# Autodesk Inventor assembly: Montiert
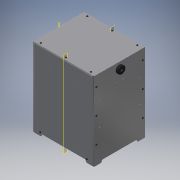
[picture p0: Inventor's stored thumbnail of the model, 180x180]
Saved by Autodesk Inventor 2018 (Build 220112000, 112)
## iProperties
Created: 2017-11-12
Part Number: Montiert
Material: Generisch
Document SubType Name: Assembly
## Documents named in this file (13)
- C:\git\RoKu-ProjectX01\Konstruktion\Montiert.iam
- C:\git\RoKu-ProjectX01\Konstruktion\Brenner.ipt
- C:\git\RoKu-ProjectX01\Konstruktion\Gegenhalter.ipt
- C:\git\RoKu-ProjectX01\Konstruktion\BrennerBrennTeil.ipt
- C:\git\RoKu-ProjectX01\Konstruktion\Back.ipt
- C:\git\RoKu-ProjectX01\Konstruktion\Seite.ipt
- C:\git\RoKu-ProjectX01\Konstruktion\Front.ipt
- C:\git\RoKu-ProjectX01\Konstruktion\Deckel.ipt
- C:\git\RoKu-ProjectX01\Konstruktion\MutterMitUScheibe.ipt
- C:\git\RoKu-ProjectX01\Konstruktion\BrennerHalter.ipt
- C:\Users\kuckal\Documents\Inventor\Content Center Files\R2018\de-DE\ISO 7380-1\ISO 7380-1 - M4 x 8.ipt
- C:\Users\kuckal\Documents\Inventor\Content Center Files\R2018\de-DE\ISO 7380-1\ISO 7380-1 - M4 x 6.ipt
- C:\Users\kuckal\Documents\Inventor\Content Center Files\R2018\de-DE\DIN EN 24 036(2)\DIN EN 24 036 - M4.ipt
## Components (65 placed, 12 different names)
1. Brenner:1 — Fluchtend:1, Fluchtend:2, Fluchtend:3, Passend:1, Passend:2, Fluchtend:4, Passend:3, Passend:4, Fluchtend:13, Fluchtend:14, Einfügen:37, Einfügen:38, Einfügen:39, Einfügen:40, Einfügen:41, Einfügen:42, Einfügen:43, Einfügen:44, Einfügen:45, Einfügen:46, Einfügen:47, Einfügen:48
2. Gegenhalter:1 — Passend:1, Passend:2, Einfügen:55, Einfügen:56, Einfügen:57, Einfügen:58, Einfügen:59, Einfügen:60, Einfügen:61, Einfügen:62, Einfügen:63, Einfügen:64, Einfügen:65, Einfügen:66
3. BrennerBrennTeil:1 — Fluchtend:4
4. Back:1 — Passend:3, Passend:4, Passend:5, Passend:6, Fluchtend:6, Fluchtend:7, Passend:7, Fluchtend:8, Fluchtend:9, Einfügen:25, Einfügen:26, Einfügen:27, Einfügen:28, Einfügen:29, Einfügen:30
5. Seite:1 — Passend:6, Fluchtend:6, Fluchtend:7, Passend:8, Fluchtend:11, Passend:9, Fluchtend:12, Passend:11, Passend:12, Passend:13, Passend:14, Einfügen:13, Einfügen:14, Einfügen:52, Einfügen:53, Einfügen:54
6. Seite:2 — Passend:7, Fluchtend:8, Fluchtend:9, Fluchtend:10, Passend:23, Passend:24, Passend:25, Passend:26, Einfügen:11, Einfügen:12, Einfügen:49, Einfügen:50, Einfügen:51
7. Front:1 — Passend:8, Fluchtend:10, Fluchtend:11, Passend:10, Einfügen:15, Einfügen:16, Einfügen:17, Einfügen:18, Einfügen:19, Einfügen:20
8. Deckel:1 — Passend:9, Fluchtend:12, Passend:10, Einfügen:31, Einfügen:32, Einfügen:33, Einfügen:34, Einfügen:35, Einfügen:36
9. MutterMitUScheibe:3 — Passend:23, Passend:24
10. MutterMitUScheibe:4 — Passend:25, Passend:26
11. MutterMitUScheibe:10 — Passend:11, Passend:12
12. MutterMitUScheibe:11 — Passend:13, Passend:14
13. BrennerHalter:1 — Fluchtend:13, Fluchtend:14
14. ISO 7380-1 M4 x 6:11 — Einfügen:11
15. ISO 7380-1 M4 x 6:12 — Einfügen:12
16. ISO 7380-1 M4 x 6:13 — Einfügen:13
17. ISO 7380-1 M4 x 6:14 — Einfügen:14
18. ISO 7380-1 M4 x 6:15 — Einfügen:15
19. ISO 7380-1 M4 x 6:16 — Einfügen:16
20. ISO 7380-1 M4 x 6:17 — Einfügen:17
21. ISO 7380-1 M4 x 6:18 — Einfügen:18
22. ISO 7380-1 M4 x 6:19 — Einfügen:19
23. ISO 7380-1 M4 x 6:20 — Einfügen:20
24. ISO 7380-1 M4 x 8:1 — Einfügen:25
25. ISO 7380-1 M4 x 8:2 — Einfügen:26
26. ISO 7380-1 M4 x 8:3 — Einfügen:27
27. ISO 7380-1 M4 x 8:4 — Einfügen:28
28. ISO 7380-1 M4 x 8:5 — Einfügen:29
29. ISO 7380-1 M4 x 8:6 — Einfügen:30
30. ISO 7380-1 M4 x 8:7 — Einfügen:31
31. ISO 7380-1 M4 x 8:8 — Einfügen:32
32. ISO 7380-1 M4 x 8:9 — Einfügen:33
33. ISO 7380-1 M4 x 8:10 — Einfügen:34
34. ISO 7380-1 M4 x 8:11 — Einfügen:35
35. ISO 7380-1 M4 x 8:12 — Einfügen:36
36. ISO 7380-1 M4 x 8:13 — Einfügen:37
37. ISO 7380-1 M4 x 8:14 — Einfügen:38
38. ISO 7380-1 M4 x 8:15 — Einfügen:39
39. ISO 7380-1 M4 x 8:16 — Einfügen:40
40. ISO 7380-1 M4 x 8:17 — Einfügen:41
41. ISO 7380-1 M4 x 8:18 — Einfügen:42
42. ISO 7380-1 M4 x 8:19 — Einfügen:43
43. ISO 7380-1 M4 x 8:20 — Einfügen:44
44. ISO 7380-1 M4 x 8:21 — Einfügen:45
45. ISO 7380-1 M4 x 8:22 — Einfügen:46
46. ISO 7380-1 M4 x 8:23 — Einfügen:47
47. ISO 7380-1 M4 x 8:24 — Einfügen:48
48. DIN EN 24036 M4:1 — Einfügen:49
49. DIN EN 24036 M4:2 — Einfügen:50
50. DIN EN 24036 M4:3 — Einfügen:51
51. DIN EN 24036 M4:4 — Einfügen:52
52. DIN EN 24036 M4:5 — Einfügen:53
53. DIN EN 24036 M4:6 — Einfügen:54
54. DIN EN 24036 M4:7 — Einfügen:55
55. DIN EN 24036 M4:8 — Einfügen:56
56. DIN EN 24036 M4:9 — Einfügen:57
57. DIN EN 24036 M4:10 — Einfügen:58
58. DIN EN 24036 M4:11 — Einfügen:59
59. DIN EN 24036 M4:12 — Einfügen:60
60. DIN EN 24036 M4:13 — Einfügen:61
61. DIN EN 24036 M4:14 — Einfügen:62
62. DIN EN 24036 M4:15 — Einfügen:63
63. DIN EN 24036 M4:16 — Einfügen:64
64. DIN EN 24036 M4:17 — Einfügen:65
65. DIN EN 24036 M4:18 — Einfügen:66
## Relationships (83: Insert 52, Mate 18, Flush 13)
- Fluchtend:1 [Flush]: Brenner:1
- Fluchtend:2 [Flush]: Brenner:1
- Fluchtend:3 [Flush]: Brenner:1
- Passend:1 [Mate] (2 mm): Brenner:1 ↔ Gegenhalter:1
- Passend:2 [Mate]: Brenner:1 ↔ Gegenhalter:1
- Fluchtend:4 [Flush]: Brenner:1 ↔ BrennerBrennTeil:1
- Passend:3 [Mate]: Brenner:1 ↔ Back:1
- Passend:4 [Mate] (-12 mm): Brenner:1 ↔ Back:1
- Passend:5 [Mate]: Back:1
- Passend:6 [Mate]: Back:1 ↔ Seite:1
- Fluchtend:6 [Flush]: Back:1 ↔ Seite:1
- Fluchtend:7 [Flush]: Back:1 ↔ Seite:1
- Passend:7 [Mate]: Back:1 ↔ Seite:2
- Fluchtend:8 [Flush]: Back:1 ↔ Seite:2
- Fluchtend:9 [Flush]: Back:1 ↔ Seite:2
- Passend:8 [Mate]: Seite:1 ↔ Front:1
- Fluchtend:10 [Flush]: Seite:2 ↔ Front:1
- Fluchtend:11 [Flush]: Seite:1 ↔ Front:1
- Passend:9 [Mate]: Seite:1 ↔ Deckel:1
- Fluchtend:12 [Flush]: Seite:1 ↔ Deckel:1
- Passend:10 [Mate]: Front:1 ↔ Deckel:1
- Passend:11 [Mate]: Seite:1 ↔ MutterMitUScheibe:10
- Passend:12 [Mate]: Seite:1 ↔ MutterMitUScheibe:10
- Passend:13 [Mate]: Seite:1 ↔ MutterMitUScheibe:11
- Passend:14 [Mate]: Seite:1 ↔ MutterMitUScheibe:11
- Passend:23 [Mate]: Seite:2 ↔ MutterMitUScheibe:3
- Passend:24 [Mate]: Seite:2 ↔ MutterMitUScheibe:3
- Passend:25 [Mate]: Seite:2 ↔ MutterMitUScheibe:4
- Passend:26 [Mate]: Seite:2 ↔ MutterMitUScheibe:4
- Fluchtend:13 [Flush]: Brenner:1 ↔ BrennerHalter:1
- Fluchtend:14 [Flush]: Brenner:1 ↔ BrennerHalter:1
- Einfügen:11 [Insert]: Seite:2 ↔ ISO 7380-1 M4 x 6:11
- Einfügen:12 [Insert]: Seite:2 ↔ ISO 7380-1 M4 x 6:12
- Einfügen:13 [Insert]: Seite:1 ↔ ISO 7380-1 M4 x 6:13
- Einfügen:14 [Insert]: Seite:1 ↔ ISO 7380-1 M4 x 6:14
- Einfügen:15 [Insert]: Front:1 ↔ ISO 7380-1 M4 x 6:15
- Einfügen:16 [Insert]: Front:1 ↔ ISO 7380-1 M4 x 6:16
- Einfügen:17 [Insert]: Front:1 ↔ ISO 7380-1 M4 x 6:17
- Einfügen:18 [Insert]: Front:1 ↔ ISO 7380-1 M4 x 6:18
- Einfügen:19 [Insert]: Front:1 ↔ ISO 7380-1 M4 x 6:19
- Einfügen:20 [Insert]: Front:1 ↔ ISO 7380-1 M4 x 6:20
- Einfügen:25 [Insert]: Back:1 ↔ ISO 7380-1 M4 x 8:1
- Einfügen:26 [Insert]: Back:1 ↔ ISO 7380-1 M4 x 8:2
- Einfügen:27 [Insert]: Back:1 ↔ ISO 7380-1 M4 x 8:3
- Einfügen:28 [Insert]: Back:1 ↔ ISO 7380-1 M4 x 8:4
- Einfügen:29 [Insert]: Back:1 ↔ ISO 7380-1 M4 x 8:5
- Einfügen:30 [Insert]: Back:1 ↔ ISO 7380-1 M4 x 8:6
- Einfügen:31 [Insert]: Deckel:1 ↔ ISO 7380-1 M4 x 8:7
- Einfügen:32 [Insert]: Deckel:1 ↔ ISO 7380-1 M4 x 8:8
- Einfügen:33 [Insert]: Deckel:1 ↔ ISO 7380-1 M4 x 8:9
- Einfügen:34 [Insert]: Deckel:1 ↔ ISO 7380-1 M4 x 8:10
- Einfügen:35 [Insert]: Deckel:1 ↔ ISO 7380-1 M4 x 8:11
- Einfügen:36 [Insert]: Deckel:1 ↔ ISO 7380-1 M4 x 8:12
- Einfügen:37 [Insert]: Brenner:1 ↔ ISO 7380-1 M4 x 8:13
- Einfügen:38 [Insert]: Brenner:1 ↔ ISO 7380-1 M4 x 8:14
- Einfügen:39 [Insert]: Brenner:1 ↔ ISO 7380-1 M4 x 8:15
- Einfügen:40 [Insert]: Brenner:1 ↔ ISO 7380-1 M4 x 8:16
- Einfügen:41 [Insert]: Brenner:1 ↔ ISO 7380-1 M4 x 8:17
- Einfügen:42 [Insert]: Brenner:1 ↔ ISO 7380-1 M4 x 8:18
- Einfügen:43 [Insert]: Brenner:1 ↔ ISO 7380-1 M4 x 8:19
- Einfügen:44 [Insert]: Brenner:1 ↔ ISO 7380-1 M4 x 8:20
- Einfügen:45 [Insert]: Brenner:1 ↔ ISO 7380-1 M4 x 8:21
- Einfügen:46 [Insert]: Brenner:1 ↔ ISO 7380-1 M4 x 8:22
- Einfügen:47 [Insert]: Brenner:1 ↔ ISO 7380-1 M4 x 8:23
- Einfügen:48 [Insert]: Brenner:1 ↔ ISO 7380-1 M4 x 8:24
- Einfügen:49 [Insert]: Seite:2 ↔ DIN EN 24036 M4:1
- Einfügen:50 [Insert]: Seite:2 ↔ DIN EN 24036 M4:2
- Einfügen:51 [Insert]: Seite:2 ↔ DIN EN 24036 M4:3
- Einfügen:52 [Insert]: Seite:1 ↔ DIN EN 24036 M4:4
- Einfügen:53 [Insert]: Seite:1 ↔ DIN EN 24036 M4:5
- Einfügen:54 [Insert]: Seite:1 ↔ DIN EN 24036 M4:6
- Einfügen:55 [Insert]: Gegenhalter:1 ↔ DIN EN 24036 M4:7
- Einfügen:56 [Insert]: Gegenhalter:1 ↔ DIN EN 24036 M4:8
- Einfügen:57 [Insert]: Gegenhalter:1 ↔ DIN EN 24036 M4:9
- Einfügen:58 [Insert]: Gegenhalter:1 ↔ DIN EN 24036 M4:10
- Einfügen:59 [Insert]: Gegenhalter:1 ↔ DIN EN 24036 M4:11
- Einfügen:60 [Insert]: Gegenhalter:1 ↔ DIN EN 24036 M4:12
- Einfügen:61 [Insert]: Gegenhalter:1 ↔ DIN EN 24036 M4:13
- Einfügen:62 [Insert]: Gegenhalter:1 ↔ DIN EN 24036 M4:14
- Einfügen:63 [Insert]: Gegenhalter:1 ↔ DIN EN 24036 M4:15
- Einfügen:64 [Insert]: Gegenhalter:1 ↔ DIN EN 24036 M4:16
- Einfügen:65 [Insert]: Gegenhalter:1 ↔ DIN EN 24036 M4:17
- Einfügen:66 [Insert]: Gegenhalter:1 ↔ DIN EN 24036 M4:18
